# Autodesk Inventor assembly: arm assembaly
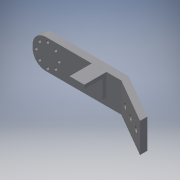
[picture p0: Inventor's stored thumbnail of the model, 180x180]
Saved by Autodesk Inventor 2019 (Build 230136000, 136)
## iProperties
Created: 2019-10-26
Part Number: arm assembaly
Document SubType Name: Assembly
Designer: User
Author: User
## Documents named in this file (3)
- C:\Robotics\CAD\2019-20_CAD\Collection\arm assembaly.iam
- C:\Robotics\CAD\2019-20_CAD\Collection\Wheel Arms.ipt
- C:\Robotics\CAD\2019-20_CAD\Collection\spring tab for on arm.ipt
## Components (2 placed, 2 different names)
1. Wheel Arms:1 — Flush:1, Mate:1, Mate:2
2. spring tab for on arm:1 — Flush:1, Mate:1, Mate:2
## Relationships (3: Mate 2, Flush 1)
- Flush:1: Wheel Arms:1 ↔ spring tab for on arm:1
- Mate:1: Wheel Arms:1 ↔ spring tab for on arm:1
- Mate:2 (12.7 mm): Wheel Arms:1 ↔ spring tab for on arm:1
